# Autodesk Inventor assembly: Assembly146-01
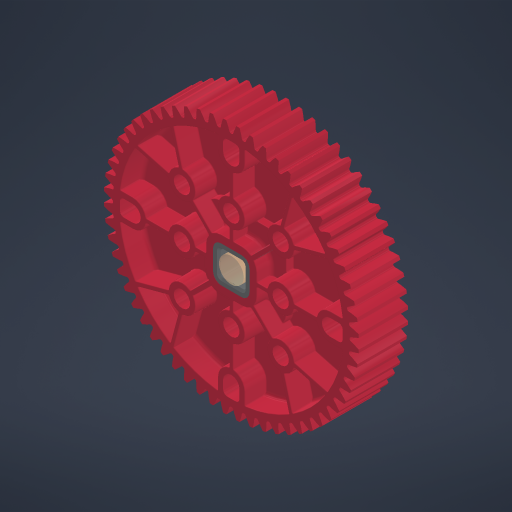
[picture p0: Inventor's stored thumbnail of the model, 512x512]
Saved by Autodesk Inventor 2024 (Build 280153000, 153)
## iProperties
Created: 2022-08-02
Part Number: Assembly146-01
Document SubType Name: Assembly
Designer: ylu12
Author: ylu12
## Documents named in this file (3)
- \\Mac\Home\Desktop\code\1599V-VRC\Cad\Motion\Gears\HS Gear\HS 60T Gear, No Insert.iam
- \\Mac\Home\Desktop\code\1599V-VRC\Cad\Motion\Gears\Reference Files\HS 60T Gear, No Insert.ipt
- \\Mac\Home\Desktop\code\1599V-VRC\Cad\Motion\Gears\HS Gear.iam
## Components (1 placed, 1 different names)
1. 60T — Flush:7, Mate:13, Mate:14
## Relationships (3: Mate 2, Flush 1)
- Flush:7: 60T
- Mate:13: 60T
- Mate:14: 60T
